# Autodesk Inventor assembly: Ball Joint
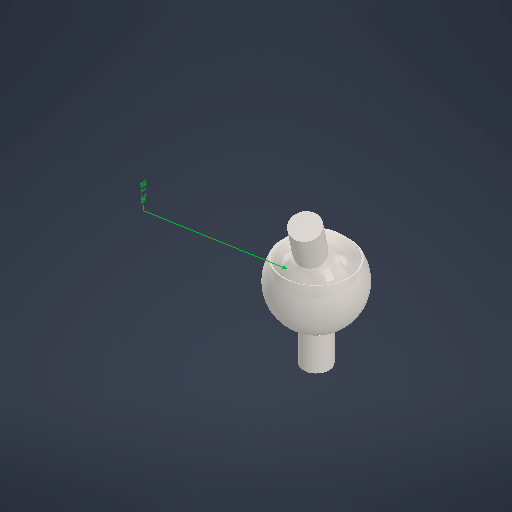
[picture p0: Inventor's stored thumbnail of the model, 512x512]
Saved by Autodesk Inventor 2026.2 (Build 302298000, 298)
## iProperties
Created: 1601-01-02
Part Number: Ball Joint
Document SubType Name: Assembly
Designer: danda
Sending System: SOLIDWORKS 2019
Last Saved Date: 1601-01-01
last saved by: admin
Author: danda
## Documents named in this file (3)
- C:\Users\danda\OneDrive\Desktop\Basics Of Mecha\Project\Ball Joint.iam
- C:\Users\danda\OneDrive\Desktop\Basics Of Mecha\Project\Ball Joint\Ball Joint\Base.ipt
- C:\Users\danda\OneDrive\Desktop\Basics Of Mecha\Project\Ball Joint\Ball Joint\Ball.ipt
## Components (2 placed, 2 different names)
1. Base-2 — Tangent:1
2. Ball-2 — Tangent:1
## Relationships (1: Tangent 1)
- Tangent:1: Base-2 ↔ Ball-2
